# Autodesk Inventor assembly: Ring_Gear_Assembly_1
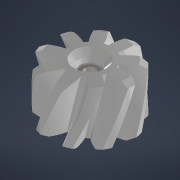
[picture p0: Inventor's stored thumbnail of the model, 180x180]
Saved by Autodesk Inventor 2021 (Build 250183000, 183)
## iProperties
Created: 2025-03-27
Part Number: Ring_Gear_Assembly_1
Document SubType Name: Assembly
Designer: rocke
Author: rocke
## Documents named in this file (3)
- C:\Users\rocke\Documents\Robot Arm IPT\Ring Gear 1\Ring_Gear_Assembly_1.iam
- C:\Users\rocke\Documents\Inventor\Content Center Files\R2021\en-US\GB_T 276-94 60000-2Z\Bearing 623-2Z GB_T 276-94.ipt
- C:\Users\rocke\Documents\Robot Arm IPT\Ring Gear 1\Planet_Gear_1.ipt
## Components (2 placed, 2 different names)
1. Spur Gear2:1 — Insert:1
2. Rolling bearing GB/T 276-1994 Type 60000-2Z 623-2Z:1 — Insert:1
## Relationships (1: Insert 1)
- Insert:1: Spur Gear2:1 ↔ Rolling bearing GB/T 276-1994 Type 60000-2Z 623-2Z:1
